# Autodesk Inventor assembly: ServoHousingAssembly
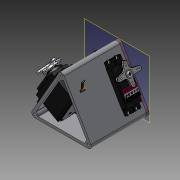
[picture p0: Inventor's stored thumbnail of the model, 180x180]
Saved by Autodesk Inventor 2014 SP1 (Build 180222100, 222)
## iProperties
Created: 2014-11-03
Part Number: ServoHousingAssembly
Document SubType Name: Assembly
Designer: rawrdong
Author: rawrdong
## Documents named in this file (4)
- C:\Users\rawrdong\Documents\GitHub\FlippityFlappity\CAD_HW\ServoHousingAssembly.iam
- C:\Users\rawrdong\Documents\GitHub\FlippityFlappity\CAD_HW\ServoHousing.ipt
- C:\Users\rawrdong\Documents\GitHub\FlippityFlappity\CAD_HW\servo-6.snapshot.1\Imported Components\Servo HS425BB\Servo HS425BB.ipt
- C:\Users\rawrdong\Documents\GitHub\FlippityFlappity\CAD_HW\ServoHousingEndPlates.ipt
## Components (5 placed, 3 different names)
1. ServoHousing:1 — Mate:1, Mate:2, Mate:3, Mate:4, Flush:1, Flush:2
2. Servo HS425BB:1 — Mate:1, Mate:2
3. Servo HS425BB:2 — Mate:3
4. Servo HS425BB:3 — Mate:4
5. ServoHousingEndPlates:1 — Flush:1, Flush:2
## Relationships (6: Mate 4, Flush 2)
- Mate:1: ServoHousing:1 ↔ Servo HS425BB:1
- Mate:2: ServoHousing:1 ↔ Servo HS425BB:1
- Mate:3: ServoHousing:1 ↔ Servo HS425BB:2
- Mate:4: ServoHousing:1 ↔ Servo HS425BB:3
- Flush:1: ServoHousing:1 ↔ ServoHousingEndPlates:1
- Flush:2: ServoHousing:1 ↔ ServoHousingEndPlates:1
